# Autodesk Inventor assembly: Y-axis assy
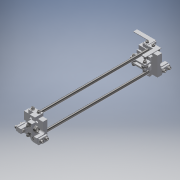
[picture p0: Inventor's stored thumbnail of the model, 180x180]
Saved by Autodesk Inventor 2018 (Build 220112000, 112)
## iProperties
Created: 2017-10-27
Part Number: Y-axis assy
Document SubType Name: Assembly
Designer: Gabriel Smolnycki
Author: Gabriel Smolnycki
## Documents named in this file (4)
- E:\planb\mechanics\Subassemblies\Y-axis assy.iam
- E:\planb\mechanics\Subassemblies\Y-axis Belt Idler assy.iam
- E:\planb\mechanics\Subassemblies\Y-axis Frame Return assy.iam
- E:\planb\mechanics\Y-axis\Y-axis Rod 8mm.ipt
## Components (4 placed, 3 different names)
1. Y-axis Belt Idler assy:1 [sub-assembly] — Insert:1, Insert:2
2. Y-axis Frame Return assy:1 [sub-assembly] — Insert:3, Insert:4
3. Y-axis Rod 8mm:1 — Insert:1, Insert:4
4. Y-axis Rod 8mm:2 — Insert:2, Insert:3
## Relationships (4: Insert 4)
- Insert:1: Y-axis Belt Idler assy:1 ↔ Y-axis Rod 8mm:1
- Insert:2: Y-axis Belt Idler assy:1 ↔ Y-axis Rod 8mm:2
- Insert:3: Y-axis Frame Return assy:1 ↔ Y-axis Rod 8mm:2
- Insert:4: Y-axis Frame Return assy:1 ↔ Y-axis Rod 8mm:1
